# Autodesk Inventor assembly: 2015 Robot
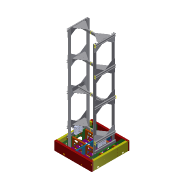
[picture p0: Inventor's stored thumbnail of the model, 180x180]
Saved by Autodesk Inventor 2015 (Build 190159000, 159)
## iProperties
Created: 2015-01-24
Part Number: 2015 Robot
Document SubType Name: Assembly
Designer: Peter
Author: Peter
## Documents named in this file (3)
- T:\FILES\FIRST-Team-1719-CAD-Team\2015 Robot CAD\2015 Robot Assembly.iam
- T:\FILES\FIRST-Team-1719-CAD-Team\2015 Robot CAD\Chassis, Wheels, and Drive Train\Chassis, Wheels, and Drive Train Assembly.iam
- T:\FILES\FIRST-Team-1719-CAD-Team\2015 Robot CAD\Two Lifters and Lifter Super Structure\Lifter Super Structure\Lifter Super Structure.iam
## Components (2 placed, 2 different names)
1. Chassis, Wheels, and Drive Train Assembly:1 [sub-assembly] — Mate:1, Mate:2, Flush:1
2. Lifter Super Structure:1 [sub-assembly] — Mate:1, Mate:2, Flush:1
## Relationships (3: Mate 2, Flush 1)
- Mate:1: Chassis, Wheels, and Drive Train Assembly:1 ↔ Lifter Super Structure:1
- Mate:2: Chassis, Wheels, and Drive Train Assembly:1 ↔ Lifter Super Structure:1
- Flush:1 (-165.1 mm): Chassis, Wheels, and Drive Train Assembly:1 ↔ Lifter Super Structure:1
